# Autodesk Inventor assembly: A2017_T4_01
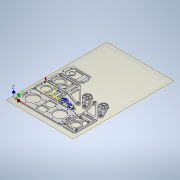
[picture p0: Inventor's stored thumbnail of the model, 180x180]
Saved by Autodesk Inventor 2020 (Build 240168000, 168)
## iProperties
Created: 2021-08-27
Part Number: A2017_T4_01
Document SubType Name: Assembly
Designer: Masato
Author: Masato
## Documents named in this file (8)
- C:\Users\naoki\Documents\Inventor\CitBrains\git_clone\SUSTAINA_ver1_0\A_T4_T2\SUSTAINA-OP\Cam\A2017_T4_01.iam
- C:\Users\naoki\Documents\Inventor\CitBrains\git_clone\SUSTAINA_ver1_0\A_T4_T2\SUSTAINA-OP\Cam\DisposableBoard.ipt
- C:\Users\naoki\Documents\Inventor\CitBrains\git_clone\SUSTAINA_ver1_0\A_T4_T2\SUSTAINA-OP\LowerBody\Ankle\Ankle_side_pitch_frame.ipt
- C:\Users\naoki\Documents\Inventor\CitBrains\git_clone\SUSTAINA_ver1_0\A_T4_T2\SUSTAINA-OP\UpperBody\Trunk\Trunk_neck_frame.ipt
- C:\Users\naoki\Documents\Inventor\CitBrains\git_clone\SUSTAINA_ver1_0\A_T4_T2\SUSTAINA-OP\UpperBody\Trunk\Trunk_shoulder_frame.ipt
- C:\Users\naoki\Documents\Inventor\CitBrains\git_clone\SUSTAINA_ver1_0\A_T4_T2\SUSTAINA-OP\UpperBody\Trunk\Trunk_shoulder_frame_MIR.ipt
- C:\Users\naoki\Documents\Inventor\CitBrains\git_clone\SUSTAINA_ver1_0\A_T4_T2\SUSTAINA-OP\UpperBody\Trunk\Trunk_waisit_frame.ipt
- C:\Users\naoki\Documents\Inventor\CitBrains\git_clone\SUSTAINA_ver1_0\A_T4_T2\SUSTAINA-OP\UpperBody\Trunk\Trunk_servo_bottom_frame.ipt
## Components (9 placed, 7 different names)
1. DisposableBoard:1 — メイト:2, メイト:1, フラッシュ:1, フラッシュ:2, フラッシュ:3, フラッシュ:5, メイト:22
2. Trunk_neck_frame:1 — メイト:6, フラッシュ:6, フラッシュ:7, メイト:16, メイト:17, 正接:2
3. Trunk_shoulder_frame:1 — メイト:9, フラッシュ:4, メイト:15, メイト:21, 正接:3, 正接:4
4. Trunk_shoulder_frame_MIR:1 — メイト:10, フラッシュ:7, メイト:17, メイト:20
5. Trunk_waisit_frame:1 — フラッシュ:3, フラッシュ:4, フラッシュ:5, フラッシュ:6, メイト:15, メイト:16, メイト:19
6. Ankle_side_pitch_frame:2 — メイト:5, メイト:19, 正接:2
7. Ankle_side_pitch_frame:1 — メイト:4, メイト:20, 正接:3
8. Trunk_servo_bottom_frame:2 — メイト:14
9. Ankle_side_pitch_frame:3 — メイト:21, メイト:22, 正接:4
## Relationships (25: Mate 15, Flush 7, Tangent 3)
- メイト:2 [Mate]: DisposableBoard:1
- メイト:1 [Mate]: DisposableBoard:1
- フラッシュ:1 [Flush]: DisposableBoard:1
- フラッシュ:2 [Flush]: DisposableBoard:1
- メイト:4 [Mate]: Ankle_side_pitch_frame:1
- メイト:5 [Mate]: Ankle_side_pitch_frame:2
- メイト:6 [Mate]: Trunk_neck_frame:1
- メイト:9 [Mate]: Trunk_shoulder_frame:1
- メイト:10 [Mate]: Trunk_shoulder_frame_MIR:1
- メイト:14 [Mate]: Trunk_servo_bottom_frame:2
- フラッシュ:3 [Flush] (2 mm): DisposableBoard:1 ↔ Trunk_waisit_frame:1
- フラッシュ:4 [Flush]: Trunk_shoulder_frame:1 ↔ Trunk_waisit_frame:1
- フラッシュ:5 [Flush] (2 mm): DisposableBoard:1 ↔ Trunk_waisit_frame:1
- フラッシュ:6 [Flush]: Trunk_neck_frame:1 ↔ Trunk_waisit_frame:1
- フラッシュ:7 [Flush]: Trunk_neck_frame:1 ↔ Trunk_shoulder_frame_MIR:1
- メイト:15 [Mate] (2.5 mm): Trunk_shoulder_frame:1 ↔ Trunk_waisit_frame:1
- メイト:16 [Mate] (2.5 mm): Trunk_neck_frame:1 ↔ Trunk_waisit_frame:1
- メイト:17 [Mate] (2.5 mm): Trunk_neck_frame:1 ↔ Trunk_shoulder_frame_MIR:1
- メイト:19 [Mate] (2.5 mm): Trunk_waisit_frame:1 ↔ Ankle_side_pitch_frame:2
- メイト:20 [Mate] (2.5 mm): Trunk_shoulder_frame_MIR:1 ↔ Ankle_side_pitch_frame:1
- メイト:21 [Mate] (2.5 mm): Trunk_shoulder_frame:1 ↔ Ankle_side_pitch_frame:3
- メイト:22 [Mate]: DisposableBoard:1 ↔ Ankle_side_pitch_frame:3
- 正接:2 [Tangent] (2.5 mm): Trunk_neck_frame:1 ↔ Ankle_side_pitch_frame:2
- 正接:3 [Tangent] (2.5 mm): Trunk_shoulder_frame:1 ↔ Ankle_side_pitch_frame:1
- 正接:4 [Tangent] (1 mm): Trunk_shoulder_frame:1 ↔ Ankle_side_pitch_frame:3
